# Autodesk Inventor assembly: DIFF_BARV2_ASM
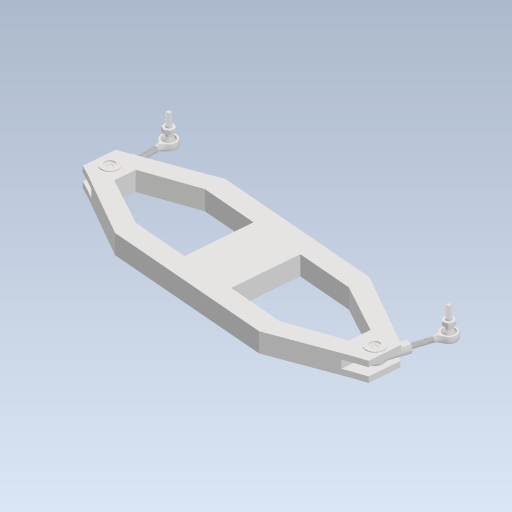
[picture p0: Inventor's stored thumbnail of the model, 512x512]
Saved by Autodesk Inventor 2023 (Build 270158000, 158)
## iProperties
Created: 2023-04-06
Part Number: DIFF_BARV2_ASM
Document SubType Name: Assembly
Designer: bugme
Author: bugme
## Documents named in this file (10)
- C:\Users\Dave\Documents\GitHub\BehrendURCMechanical\CAD\Chassis V3\Diff Bar\DIFF_BARV2_ASM.iam
- C:\Users\Dave\Documents\GitHub\BehrendURCMechanical\CAD\Chassis V3\Diff Bar\Diff_BarV2.ipt
- C:\Users\Dave\Documents\GitHub\BehrendURCMechanical\CAD\Chassis V3\Diff Bar\60645K211_Ball Joint Linkage.ipt
- C:\Users\Dave\Documents\GitHub\BehrendURCMechanical\CAD\Chassis V3\Diff Bar\59915K481_Corrosion-Resistant Ball Joint Rod End.ipt
- C:\Users\Dave\Documents\GitHub\BehrendURCMechanical\CAD\Chassis V3\Diff Bar\98381A505_Dowel Pin.ipt
- C:\Users\Dave\Documents\GitHub\BehrendURCMechanical\CAD\Chassis V3\Diff Bar\1293N114_Self-Aligning Flanged Ball Bearing.ipt
- C:\Users\Dave\Documents\GitHub\BehrendURCMechanical\CAD\Chassis V3\Diff Bar\60645K211_Ball Joint Linkage_MIR.ipt
- C:\Users\Dave\Documents\GitHub\BehrendURCMechanical\CAD\Chassis V3\Diff Bar\59915K481_Corrosion-Resistant Ball Joint Rod End_MIR.ipt
- C:\Users\Dave\Documents\GitHub\BehrendURCMechanical\CAD\Chassis V3\Diff Bar\98381A505_Dowel Pin_MIR.ipt
- C:\Users\Dave\Documents\GitHub\BehrendURCMechanical\CAD\Chassis V3\Diff Bar\1293N114_Self-Aligning Flanged Ball Bearing_MIR.ipt
## Components (9 placed, 9 different names)
1. Diff_BarV2:1 — Insert:5, Flush:1, Insert:9
2. 60645K211_Ball Joint Linkage:1 — Insert:4
3. 59915K481_Corrosion-Resistant Ball Joint Rod End:1 — Insert:3, Insert:4
4. 98381A505_Dowel Pin:1 — Insert:2, Insert:3
5. 1293N114_Self-Aligning Flanged Ball Bearing:1 — Insert:2, Insert:5
6. 60645K211_Ball Joint Linkage_MIR:1 — Insert:6
7. 59915K481_Corrosion-Resistant Ball Joint Rod End_MIR:1 — Insert:6, Insert:7
8. 98381A505_Dowel Pin_MIR:1 — Insert:7, Insert:8
9. 1293N114_Self-Aligning Flanged Ball Bearing_MIR:1 — Insert:8, Insert:9
## Relationships (9: Insert 8, Flush 1)
- Insert:2: 98381A505_Dowel Pin:1 ↔ 1293N114_Self-Aligning Flanged Ball Bearing:1
- Insert:3: 59915K481_Corrosion-Resistant Ball Joint Rod End:1 ↔ 98381A505_Dowel Pin:1
- Insert:4: 60645K211_Ball Joint Linkage:1 ↔ 59915K481_Corrosion-Resistant Ball Joint Rod End:1
- Insert:5: Diff_BarV2:1 ↔ 1293N114_Self-Aligning Flanged Ball Bearing:1
- Flush:1 (-155.303 mm): Diff_BarV2:1
- Insert:6: 60645K211_Ball Joint Linkage_MIR:1 ↔ 59915K481_Corrosion-Resistant Ball Joint Rod End_MIR:1
- Insert:7: 59915K481_Corrosion-Resistant Ball Joint Rod End_MIR:1 ↔ 98381A505_Dowel Pin_MIR:1
- Insert:8: 98381A505_Dowel Pin_MIR:1 ↔ 1293N114_Self-Aligning Flanged Ball Bearing_MIR:1
- Insert:9: Diff_BarV2:1 ↔ 1293N114_Self-Aligning Flanged Ball Bearing_MIR:1
